# Autodesk Inventor assembly: Butterfly Drive Base
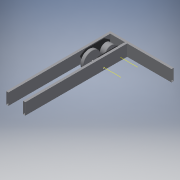
[picture p0: Inventor's stored thumbnail of the model, 180x180]
Saved by Autodesk Inventor 2019 (Build 230136000, 136)
## iProperties
Created: 2019-10-19
Part Number: Butterfly Drive Base
Document SubType Name: Assembly
Designer: Mark
Author: Mark
## Documents named in this file (6)
- C:\Users\Mark\Desktop\7738 Helion Engineering\7738-CAD-prep\Butterfly drive\Butterfly Drive Base.iam
- C:\Users\Mark\Desktop\7738 Helion Engineering\7738-CAD-prep\Butterfly drive\Butterfly Drive Module.iam
- C:\Users\Mark\Desktop\7738 Helion Engineering\7738-CAD-prep\Butterfly drive\Side Extrusion.ipt
- C:\Users\Mark\Desktop\7738 Helion Engineering\7738-CAD-prep\Butterfly drive\Module Plate 1.ipt
- C:\Users\Mark\Desktop\7738 Helion Engineering\7738-CAD-prep\Butterfly drive\Side Extrusion 2.ipt
- C:\Users\Mark\Desktop\7738 Helion Engineering\7738-CAD-prep\Butterfly drive\Back Extrusion 1.ipt
## Components (4 placed, 4 different names)
1. Butterfly Drive Module:1 [sub-assembly] — Rotational:1, Rotational:2
2. Side Extrusion:1 — Rotational:1, Angle:1
3. Side Extrusion 2:1 — Rotational:2, Angle:1, Rigid:1
4. Back Extrusion 1:1 — Rigid:1
## Relationships (4: RevoluteJoint 2, Angle 1, WeldJoint 1)
- Rotational:1 [RevoluteJoint] (5 mm): Butterfly Drive Module:1 ↔ Side Extrusion:1
- Rotational:2 [RevoluteJoint] (-5 mm): Butterfly Drive Module:1 ↔ Side Extrusion 2:1
- Angle:1 (0 deg): Side Extrusion:1 ↔ Side Extrusion 2:1
- Rigid:1 [WeldJoint]: Side Extrusion 2:1 ↔ Back Extrusion 1:1
